# Autodesk Inventor assembly: toss up A bot one motor on gearbox
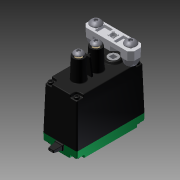
[picture p0: Inventor's stored thumbnail of the model, 180x180]
Saved by Autodesk Inventor 2014 SP1 (Build 180222100, 222)
## iProperties
Created: 2013-08-29
Part Number: toss up A bot one motor on gearbox
Document SubType Name: Assembly
Designer: Ryan
Sending System: SolidWorks 2013
Last Author: Ryan
Author: Ryan
## Documents named in this file (7)
- C:\Users\Ryan\Desktop\sw\toss up 1st A bot\inventor drive\toss up A bot one motor on gearbox.iam
- C:\Users\Ryan\Desktop\sw\lib\Aperture VEX CAD Library\Bearing Blocks\bearing block.ipt
- C:\Users\Ryan\Desktop\sw\lib\Super Sonic Sparks VEX CAD Library\Motors & Sensors\2-wire motor 393-without wire.iam
- C:\Users\Ryan\Desktop\sw\lib\Aperture VEX CAD Library\Hardware\6-32\6-32_.250.ipt
- C:\Users\Ryan\Desktop\sw\lib\Aperture VEX CAD Library\Hardware\8-32\8-32_.500.ipt
- C:\Users\Ryan\Desktop\sw\lib\Aperture VEX CAD Library\Hardware\8-32\8-32 nylock.ipt
- C:\Users\Ryan\Desktop\sw\lib\Aperture VEX CAD Library\Spacers\spacer-0500-0125.ipt
## Components (9 placed, 6 different names)
1. bearing block:1 — Mate:1, Mate:2, Mate:3, Mate:4, Mate:6, Mate:8, Mate:9, Mate:10, Mate:15, Flush:1, Angle:1
2. 6-32_-250:1 — Mate:12, Mate:13
3. 6-32_-250:2 — Mate:11, Mate:14
4. 8-32_-500:1 — Mate:1, Mate:2, Mate:7
5. 8-32_-500:2 — Mate:3, Mate:4, Mate:5
6. 8-32 nylock:1 — Mate:5, Mate:6
7. 8-32 nylock:2 — Mate:7, Mate:8
8. spacer-0500-0125:1 — Mate:9, Mate:10
9. 2-wire motor 393-without wire:2 [sub-assembly] — Mate:11, Mate:12, Mate:13, Mate:14, Mate:15, Flush:1, Angle:1
## Relationships (17: Mate 15, Flush 1, Angle 1)
- Mate:1: bearing block:1 ↔ 8-32_-500:1
- Mate:2 (1.1684 mm): bearing block:1 ↔ 8-32_-500:1
- Mate:3 (1.1684 mm): bearing block:1 ↔ 8-32_-500:2
- Mate:4: bearing block:1 ↔ 8-32_-500:2
- Mate:5: 8-32_-500:2 ↔ 8-32 nylock:1
- Mate:6: bearing block:1 ↔ 8-32 nylock:1
- Mate:7: 8-32_-500:1 ↔ 8-32 nylock:2
- Mate:8: bearing block:1 ↔ 8-32 nylock:2
- Mate:9: bearing block:1 ↔ spacer-0500-0125:1
- Mate:10: bearing block:1 ↔ spacer-0500-0125:1
- Mate:11: 6-32_-250:2 ↔ 2-wire motor 393-without wire:2
- Mate:12: 6-32_-250:1 ↔ 2-wire motor 393-without wire:2
- Mate:13 (1.1684 mm): 6-32_-250:1 ↔ 2-wire motor 393-without wire:2
- Mate:14 (1.1684 mm): 6-32_-250:2 ↔ 2-wire motor 393-without wire:2
- Mate:15: bearing block:1 ↔ 2-wire motor 393-without wire:2
- Flush:1: bearing block:1 ↔ 2-wire motor 393-without wire:2
- Angle:1 (90 deg): bearing block:1 ↔ 2-wire motor 393-without wire:2
## Named parameters: metal = 1.1684 mm
